# Autodesk Inventor assembly: Full Ring
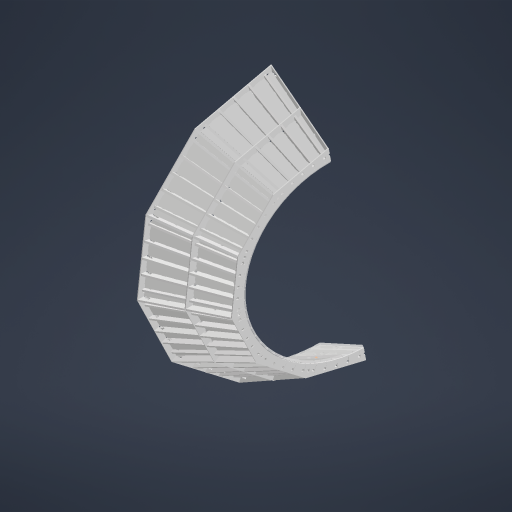
[picture p0: Inventor's stored thumbnail of the model, 512x512]
Saved by Autodesk Inventor 2023 (Build 270158000, 158)
## iProperties
Created: 2022-06-13
Part Number: Full Ring
Document SubType Name: Assembly
Designer: FizzyApple12
Author: FizzyApple12
## Documents named in this file (2)
- C:\Users\FizzyApple12\Desktop\WaccaController\Wacca Controller\Half Ring\Half Ring.iam
- C:\Users\FizzyApple12\Desktop\WaccaController\Wacca Controller\Touch Segment\Touch Segment.iam
## Components (6 placed, 1 different names)
1. Touch Segment:1 [sub-assembly] — Mate:1, Mate:6, Mate:7, Mate:8, Mate:9
2. Touch Segment:2 [sub-assembly] — Mate:1, Mate:2, Mate:6
3. Touch Segment:3 [sub-assembly] — Mate:2, Mate:3, Mate:7, Mate:10
4. Touch Segment:4 [sub-assembly] — Mate:3, Mate:4, Mate:8
5. Touch Segment:5 [sub-assembly] — Mate:4, Mate:5, Mate:9
6. Touch Segment:6 [sub-assembly] — Mate:5, Mate:10
## Relationships (10: Mate 10)
- Mate:1: Touch Segment:1 ↔ Touch Segment:2
- Mate:2: Touch Segment:2 ↔ Touch Segment:3
- Mate:3: Touch Segment:3 ↔ Touch Segment:4
- Mate:4: Touch Segment:4 ↔ Touch Segment:5
- Mate:5: Touch Segment:5 ↔ Touch Segment:6
- Mate:6: Touch Segment:1 ↔ Touch Segment:2
- Mate:7: Touch Segment:1 ↔ Touch Segment:3
- Mate:8: Touch Segment:1 ↔ Touch Segment:4
- Mate:9: Touch Segment:1 ↔ Touch Segment:5
- Mate:10: Touch Segment:3 ↔ Touch Segment:6
